# Autodesk Inventor assembly: final_aassembly
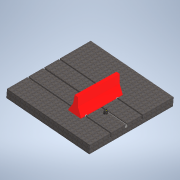
[picture p0: Inventor's stored thumbnail of the model, 180x180]
Saved by Autodesk Inventor 2022 (Build 260153000, 153)
## iProperties
Created: 2021-11-07
Part Number: final_aassembly
Document SubType Name: Assembly
Designer: kibandi
Author: kibandi
## Documents named in this file (4)
- C:\academics\YEAR 4\4.2\DOMS II\DOMS II projects\mechanical design\final_aassembly.iam
- C:\academics\YEAR 4\4.2\DOMS II\DOMS II projects\mechanical design\Pavement.ipt
- C:\academics\YEAR 4\4.2\DOMS II\DOMS II projects\mechanical design\jersey_wheels_assembly.iam
- C:\academics\YEAR 4\4.2\DOMS II\DOMS II projects\mechanical design\pneumatic_cylinder_assembly.iam
## Components (3 placed, 3 different names)
1. Pavement:1 — Mate:1, Mate:2, Mate:3
2. jersey_wheels_assembly:1 [sub-assembly] — Mate:4
3. pneumatic_cylinder_assembly:1 [sub-assembly] — Mate:1, Mate:2, Mate:3, Mate:4
## Relationships (4: Mate 4)
- Mate:1: Pavement:1 ↔ pneumatic_cylinder_assembly:1
- Mate:2: Pavement:1 ↔ pneumatic_cylinder_assembly:1
- Mate:3: Pavement:1 ↔ pneumatic_cylinder_assembly:1
- Mate:4: jersey_wheels_assembly:1 ↔ pneumatic_cylinder_assembly:1
